# Autodesk Inventor assembly: PMaxFamily
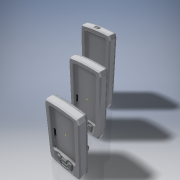
[picture p0: Inventor's stored thumbnail of the model, 180x180]
Saved by Autodesk Inventor 2018 (Build 220112000, 112)
## iProperties
Created: 2019-05-29
Part Number: PMaxFamily
Document SubType Name: Assembly
Designer: Ash
Author: Ash
## Documents named in this file (5)
- C:\Autodesk\Skills 2019 Nationals\Competition\PMDay2\PMaxFamily.iam
- C:\Autodesk\Skills 2019 Nationals\Competition\PMDay2\PMax4.iam
- C:\Autodesk\Skills 2019 Nationals\Competition\PMDay2\PMax6.iam
- C:\Autodesk\Skills 2019 Nationals\Competition\PMDay2\PMax8.iam
- C:\Autodesk\Skills 2019 Nationals\Competition\PMDay2\Part29.ipt
## Components (4 placed, 4 different names)
1. PMax4:1 [sub-assembly] — Mate:3
2. PMax6:1 [sub-assembly] — Mate:2
3. PMax8:1 [sub-assembly] — Mate:1
4. Part29:1 — Mate:1, Mate:2, Mate:3
## Relationships (3: Mate 3)
- Mate:1: PMax8:1 ↔ Part29:1
- Mate:2: PMax6:1 ↔ Part29:1
- Mate:3: PMax4:1 ↔ Part29:1
